# Autodesk Inventor assembly: DelrinX-Wheel-Bottom
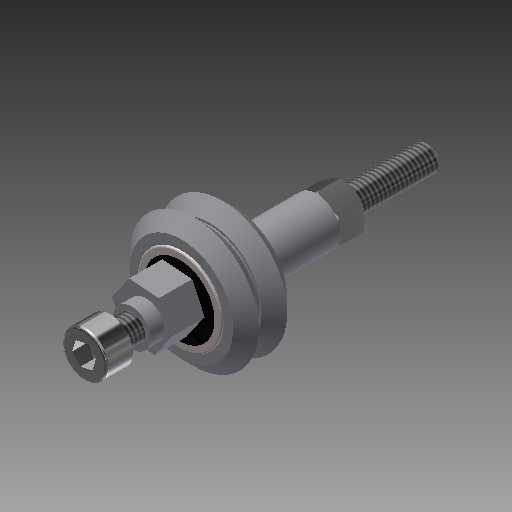
[picture p0: Inventor's stored thumbnail of the model, 512x512]
Saved by Autodesk Inventor 2017 (Build 210142000, 142)
## iProperties
Created: 2016-07-20
Part Number: DelrinX-Wheel-Bottom
Document SubType Name: Assembly
Designer: User
Author: User
## Documents named in this file (7)
- C:\All INVENTOR\SL-Inventor\SL-Beast 3D Printer\DelrinX-Wheel-Bottom.iam
- C:\All INVENTOR\SL-Inventor\SL-Beast 3D Printer\DelrinWheel.iam
- Delrin Wheel.iam
- C:\All INVENTOR\SL-Inventor\SL-Beast 3D Printer\Long-Spacer.ipt
- C:\All INVENTOR\SL-Inventor\SL-Beast 3D Printer\ANSI B18.3.1M - M5x0.8 x 60NEW.ipt
- C:\All INVENTOR\SL-Inventor\SL-Beast 3D Printer\en-US\ANSI B 18.2.4.1 M(1)\ANSI B 18.2.4.1 M - M5 x 0.8Style 2.ipt
- C:\All INVENTOR\SL-Inventor\SL-Beast 3D Printer\Eccentric Spacer.ipt
## Components (5 placed, 5 different names)
1. Delrin Wheel:1 [sub-assembly] — Mate:1, Mate:2, Mate:4
2. Long-Spacer:1 — Insert:1
3. Forged Socket Head Cap Screw - Metric M5x0.8 x 60:1 — Mate:1, Mate:2, Mate:3
4. Hex Nut Metric M5 x 0.8:1 — Insert:1
5. Eccentric Spacer:1 — Mate:3, Mate:4
## Relationships (5: Mate 4, Insert 1)
- Mate:1: Delrin Wheel:1 ↔ Forged Socket Head Cap Screw - Metric M5x0.8 x 60:1
- Insert:1: Long-Spacer:1 ↔ Hex Nut Metric M5 x 0.8:1
- Mate:2 (13 mm): Delrin Wheel:1 ↔ Forged Socket Head Cap Screw - Metric M5x0.8 x 60:1
- Mate:3: Forged Socket Head Cap Screw - Metric M5x0.8 x 60:1 ↔ Eccentric Spacer:1
- Mate:4: Delrin Wheel:1 ↔ Eccentric Spacer:1
